# Autodesk Inventor assembly: ASY MSC 010 cone
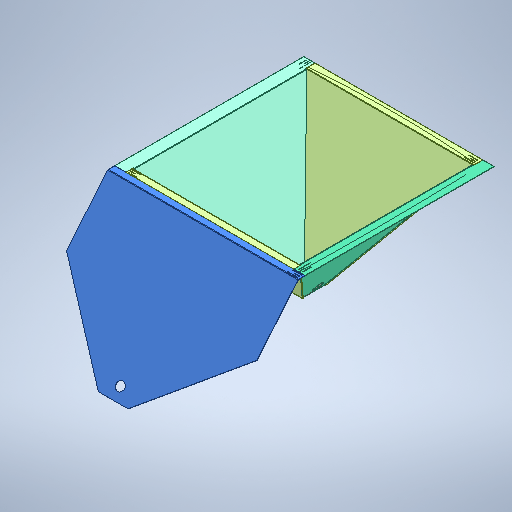
[picture p0: Inventor's stored thumbnail of the model, 512x512]
Saved by Autodesk Inventor 2025 (Build 290162010, 162A)
## iProperties
Created: 2024-05-19
Part Number: ASY MSC 010 cone
Document SubType Name: Assembly
Designer: admin
Mass: 24706.5 g
Surface Area: 124528 cm^2
Volume: 24706.5 cm^3
Density: 1 g/cm^3
Stock Number: ASY МОО 010 конус
Author: admin
## Documents named in this file (8)
- C:\Users\pokla\Documents\Inventor\Отстойник осветлитель\Manturovo_Se-clar-Gleb\ASY MSC 010 cone.iam
- C:\Users\pokla\Documents\Inventor\Отстойник осветлитель\Manturovo_Se-clar-Gleb\конус\MSC 014 cone IN right board.ipt
- C:\Users\pokla\Documents\Inventor\Отстойник осветлитель\Manturovo_Se-clar-Gleb\конус\MSC 011 cone IN bottom.ipt
- C:\Users\pokla\Documents\Inventor\Отстойник осветлитель\Manturovo_Se-clar-Gleb\конус\MSC 013 cone IN left board.ipt
- C:\Users\pokla\Documents\Inventor\Отстойник осветлитель\Manturovo_Se-clar-Gleb\конус\MSC 012 cone IN back.ipt
- C:\Users\pokla\Documents\Inventor\Отстойник осветлитель\Manturovo_Se-clar-Gleb\конус\MSC 019 cone sketch.ipt
- C:\Users\pokla\Documents\Inventor\Отстойник осветлитель\Manturovo_Se-clar-Gleb\конус\MSC 015 cone IN bow.ipt
- C:\Users\pokla\Documents\Inventor\Отстойник осветлитель\Manturovo_Se-clar-Gleb\конус\MSC 016 cone exit back.ipt
## Components (7 placed, 7 different names)
1. MSC 019 cone sketch.ipt:1 — Flush:8, Flush:9, Mate:1
2. MSC 012 cone IN back.ipt:1 — Flush:6, Flush:10, Mate:2, Flush:12
3. MSC 011 cone IN bottom.ipt:1 — Flush:4, Flush:5, Flush:11
4. MSC 014 cone IN right board.ipt:1 — Flush:12, Flush:13, Flush:15
5. MSC 013 cone IN left board.ipt:1 — Mate:4, Flush:14, Mate:5
6. MSC 015 cone IN bow.ipt:1 — Mate:3, Mate:6, Flush:16, Flush:17, Rigid:1
7. MSC 016 cone exit back.ipt:1 — Rigid:1
## Relationships (20: Flush 13, Mate 6, WeldJoint 1)
- Flush:4: MSC 011 cone IN bottom.ipt:1
- Flush:5: MSC 011 cone IN bottom.ipt:1
- Flush:6: MSC 012 cone IN back.ipt:1
- Flush:8: MSC 019 cone sketch.ipt:1
- Flush:9: MSC 019 cone sketch.ipt:1
- Mate:1: MSC 019 cone sketch.ipt:1
- Flush:10: MSC 012 cone IN back.ipt:1
- Mate:2: MSC 012 cone IN back.ipt:1
- Flush:11 (-230 mm): MSC 011 cone IN bottom.ipt:1
- Mate:3: MSC 015 cone IN bow.ipt:1
- Flush:12: MSC 012 cone IN back.ipt:1 ↔ MSC 014 cone IN right board.ipt:1
- Flush:13: MSC 014 cone IN right board.ipt:1
- Mate:4: MSC 013 cone IN left board.ipt:1
- Flush:14: MSC 013 cone IN left board.ipt:1
- Mate:5: MSC 013 cone IN left board.ipt:1
- Flush:15: MSC 014 cone IN right board.ipt:1
- Mate:6: MSC 015 cone IN bow.ipt:1
- Flush:16: MSC 015 cone IN bow.ipt:1
- Flush:17: MSC 015 cone IN bow.ipt:1
- Rigid:1 [WeldJoint]: MSC 015 cone IN bow.ipt:1 ↔ MSC 016 cone exit back.ipt:1
